# Autodesk Inventor assembly: Tape Measure Bracket Assembly V4
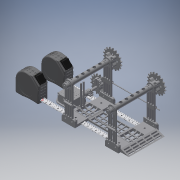
[picture p0: Inventor's stored thumbnail of the model, 180x180]
Saved by Autodesk Inventor 2019 (Build 230136000, 136)
## iProperties
Created: 2018-11-08
Part Number: Tape Measure Bracket Assembly V4
Document SubType Name: Assembly
Designer: Ashley
Author: Ashley
## Documents named in this file (16)
- C:\Users\Ashley\Desktop\repositories\design\inventor\2018-2019\Tape Measure Braket\Version Four\Tape Measure Bracket Assembly V4.iam
- C:\Users\Ashley\Desktop\repositories\design\inventor\2018-2019\Tape Measure Braket\Version Four\Bracket Bottom V4.ipt
- C:\Users\Ashley\Desktop\repositories\design\inventor\2018-2019\Tape Measure Braket\Tape Measure\Tape Measure Edited.iam
- C:\Users\Ashley\Desktop\repositories\design\inventor\2018-2019\Tape Measure Braket\Version Four\Side V4.ipt
- C:\Users\Ashley\Desktop\repositories\design\inventor\Imported Components\goBilda\Bearing6mmID.ipt
- C:\Users\Ashley\Desktop\repositories\design\inventor\2018-2019\Tape Measure Braket\Version Four\SpinnerV4.ipt
- C:\Users\Ashley\Desktop\repositories\design\inventor\Imported Components\goBilda\Collar6mm\SetScrewCollar6mmboreassembly.iam
- C:\Users\Ashley\Desktop\repositories\design\inventor\2018-2019\Tape Measure Braket\Finished Parts\2mmAxel.ipt
- C:\Users\Ashley\Desktop\repositories\design\inventor\Imported Components\goBilda\CampingHub\ClampingHub assembly.iam
- C:\Users\Ashley\Desktop\repositories\design\inventor\Imported Components\goBilda\8mmPlasticPitchSproket.ipt
- C:\Users\Ashley\Desktop\repositories\design\inventor\2018-2019\Tape Measure Braket\Version Two\Braket Top V2.ipt
- C:\Users\Ashley\Desktop\repositories\design\inventor\Imported Components\REV\Motors and Servos\Rev_Servo.iam
- C:\Users\Ashley\Desktop\repositories\design\inventor\2018-2019\Tape Measure Braket\Version Three\Servo Locks V3.ipt
- C:\Users\Ashley\Desktop\repositories\design\inventor\Imported Components\goBilda\Servo To Shaft\ServoToShaftCoupler.iam
- C:\Users\Ashley\Desktop\repositories\design\inventor\Imported Components\goBilda\DShaft40mm.ipt
- C:\Users\Ashley\Desktop\repositories\design\inventor\Imported Components\goBilda\DShaft30mm.ipt
## Components (40 placed, 27 different names)
1. Bracket Bottom — Mate:4, Mate:5, Mate:6, Mate:7, Mate:10, Mate:13, Mate:14
2. Tape Measure Right [sub-assembly]
3. Tape Measure Left [sub-assembly]
4. Back Right Side — Mate:14
5. Front Right Side — Mate:13
6. Front Left Side — Insert:3, Insert:10
7. Back Right Bearing — Insert:39
8. Front Right Bearing — Insert:38
9. Front Left Beaing — Insert:3, Insert:41
10. Front Left BEaring — Insert:23, Insert:40
11. Back Spinner — Insert:46
12. Front Spinner — Insert:51
13. Back Right Collar [sub-assembly]
14. Left axel — Insert:10
15. Right Axel
16. Back Sproket — Insert:42
17. Back Clamping Hub [sub-assembly] — Insert:42, Insert:52
18. Side V4:4 — Insert:23, Mate:10
19. Braket Top V2:1 — Mate:5
20. Braket Top V2:2 — Mate:4
21. Braket Top V2:3
22. Braket Top V2:4
23. Rev_Servo:1 [sub-assembly] — Mate:8, Insert:24
24. Servo Locks V3:1 — Mate:7, Mate:8
25. Servo Locks V3:2 — Mate:6
26. ServoToShaftCoupler:1 [sub-assembly] — Insert:24, Insert:25
27. DShaft40mm:1 — Insert:25, Insert:27
28. 8mmPlasticPitchSproket:3 — Insert:28
29. ClampingHub assembly:3 [sub-assembly] — Insert:27, Insert:28
30. DShaft30mm:2 — Insert:39, Insert:44
31. DShaft30mm:3 — Insert:41, Insert:50, Insert:51, Insert:52
32. DShaft30mm:4 — Insert:40, Insert:45, Insert:46, Insert:53
33. DShaft30mm:5 — Insert:38, Insert:47, Insert:48
34. SetScrewCollar6mmboreassembly:8 [sub-assembly] — Insert:44
35. 8mmPlasticPitchSproket:4
36. ClampingHub assembly:4 [sub-assembly] — Insert:53
37. SetScrewCollar6mmboreassembly:11 [sub-assembly] — Insert:47
38. SetScrewCollar6mmboreassembly:12 [sub-assembly] — Insert:45
39. SetScrewCollar6mmboreassembly:13 [sub-assembly] — Insert:48
40. SetScrewCollar6mmboreassembly:14 [sub-assembly] — Insert:50
## Relationships (31: Insert 22, Mate 9)
- Insert:3: Front Left Side ↔ Front Left Beaing
- Insert:10 (-30 mm): Front Left Side ↔ Left axel
- Insert:23: Front Left BEaring ↔ Side V4:4
- Mate:4: Bracket Bottom ↔ Braket Top V2:2
- Mate:5: Bracket Bottom ↔ Braket Top V2:1
- Mate:6: Bracket Bottom ↔ Servo Locks V3:2
- Mate:7: Bracket Bottom ↔ Servo Locks V3:1
- Mate:8: Rev_Servo:1 ↔ Servo Locks V3:1
- Insert:24 (-3.5 mm): Rev_Servo:1 ↔ ServoToShaftCoupler:1
- Insert:25 (30 mm): ServoToShaftCoupler:1 ↔ DShaft40mm:1
- [Insert] (-1 mm): 8mmPlasticPitchSproket:3 ↔ ClampingHub assembly:3
- Insert:27 (3 mm): DShaft40mm:1 ↔ ClampingHub assembly:3
- Insert:28 (-1 mm): 8mmPlasticPitchSproket:3 ↔ ClampingHub assembly:3
- Mate:10: Bracket Bottom ↔ Side V4:4
- Mate:13: Bracket Bottom ↔ Front Right Side
- Mate:14: Bracket Bottom ↔ Back Right Side
- Insert:38 (15 mm): Front Right Bearing ↔ DShaft30mm:5
- Insert:39 (15 mm): Back Right Bearing ↔ DShaft30mm:2
- Insert:40 (15 mm): Front Left BEaring ↔ DShaft30mm:4
- Insert:41 (15 mm): Front Left Beaing ↔ DShaft30mm:3
- [Mate]: 8mmPlasticPitchSproket:4 ↔ ClampingHub assembly:4
- Insert:42: Back Sproket ↔ Back Clamping Hub
- Insert:44 (-6.8 mm): DShaft30mm:2 ↔ SetScrewCollar6mmboreassembly:8
- Insert:45 (-14.6 mm): DShaft30mm:4 ↔ SetScrewCollar6mmboreassembly:12
- Insert:46 (-6 mm): Back Spinner ↔ DShaft30mm:4
- Insert:47 (-9 mm): DShaft30mm:5 ↔ SetScrewCollar6mmboreassembly:11
- Insert:48 (-14.6 mm): DShaft30mm:5 ↔ SetScrewCollar6mmboreassembly:13
- Insert:50 (-14.5 mm): DShaft30mm:3 ↔ SetScrewCollar6mmboreassembly:14
- Insert:51 (-6 mm): Front Spinner ↔ DShaft30mm:3
- Insert:52 (-9 mm): Back Clamping Hub ↔ DShaft30mm:3
- Insert:53 (-9 mm): DShaft30mm:4 ↔ ClampingHub assembly:4
## Named parameters: d46_d26_d25 = -1 mm, d76_d75 = 0 mm
